# Autodesk Inventor assembly: lower link
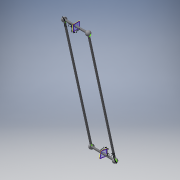
[picture p0: Inventor's stored thumbnail of the model, 180x180]
Saved by Autodesk Inventor 2016 (Build 200138000, 138)
## iProperties
Created: 2016-04-21
Part Number: lower link
Document SubType Name: Assembly
Designer: Sam
Author: Sam
## Documents named in this file (3)
- C:\Users\Sam\Documents\Three Dees\Pen Plotter\lower link assembly\lower link.iam
- C:\Users\Sam\Documents\Three Dees\Pen Plotter\lower link assembly\crossbar.ipt
- C:\Users\Sam\Documents\Three Dees\Pen Plotter\lower link assembly\longbar.ipt
## Components (4 placed, 2 different names)
1. crossbar:1 — Tangent:1, Tangent:3
2. longbar:1 — Tangent:1, Tangent:2
3. crossbar:2 — Tangent:2, Tangent:4
4. longbar:2 — Tangent:3, Tangent:4
## Relationships (4: Tangent 4)
- Tangent:1: crossbar:1 ↔ longbar:1
- Tangent:2: longbar:1 ↔ crossbar:2
- Tangent:3: crossbar:1 ↔ longbar:2
- Tangent:4: crossbar:2 ↔ longbar:2
